# Autodesk Inventor assembly: Pulley_Assembly
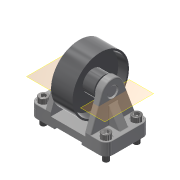
[picture p0: Inventor's stored thumbnail of the model, 180x180]
Saved by Autodesk Inventor 2022 Beta2 (Build 260130000, 130) ContinuousBuild 0
## iProperties
Created: 2016-03-03
Part Number: Pulley_Assembly
Document SubType Name: Assembly
Designer: jmacmillan
Mass: 982.528 g
Surface Area: 279.092 cm^2
Volume: 125.163 cm^3
Density: 7.85 g/cm^3
Author: jmacmillan
## Documents named in this file (6)
- C:\Autodesk Inventor 2021 Intro Practice Files\Presentation\Wheel_Assembly.iam
- C:\Autodesk Inventor 2021 Intro Practice Files\Presentation\Plate.ipt
- C:\Autodesk Inventor 2021 Intro Practice Files\Presentation\Bracket.ipt
- C:\Autodesk Inventor 2021 Intro Practice Files\Presentation\Axle.ipt
- C:\Autodesk Inventor 2021 Intro Practice Files\Presentation\Wheel.ipt
- C:\Autodesk Inventor 2021 Intro Practice Files\Presentation\M10 x 35.ipt
## Components (9 placed, 5 different names)
1. Plate:1 — Rigid:1, Rigid:2
2. Bracket:1 — Rigid:1, Angle:1, Rigid:3, Rigid:6
3. Bracket:2 — Rigid:2, Cylindrical:1, Rigid:4, Rigid:5
4. Axle:1 — Cylindrical:1, Flush:1, Angle:1, Rotational:1
5. Wheel:1 — Rotational:1
6. M10 x 35:1 — Rigid:3
7. M10 x 35:2 — Rigid:6
8. M10 x 35:3 — Rigid:4
9. M10 x 35:4 — Rigid:5
## Relationships (10: WeldJoint 6, CylindricalJoint 1, Flush 1, Angle 1, RevoluteJoint 1)
- Rigid:1 [WeldJoint]: Plate:1 ↔ Bracket:1
- Rigid:2 [WeldJoint]: Plate:1 ↔ Bracket:2
- Cylindrical:1: Bracket:2 ↔ Axle:1
- Flush:1: Axle:1
- Angle:1 (0 deg): Bracket:1 ↔ Axle:1
- Rotational:1 [RevoluteJoint]: Axle:1 ↔ Wheel:1
- Rigid:3 [WeldJoint]: Bracket:1 ↔ M10 x 35:1
- Rigid:6 [WeldJoint]: Bracket:1 ↔ M10 x 35:2
- Rigid:4 [WeldJoint]: Bracket:2 ↔ M10 x 35:3
- Rigid:5 [WeldJoint]: Bracket:2 ↔ M10 x 35:4
